# Autodesk Inventor assembly: HorizontalBit
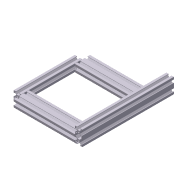
[picture p0: Inventor's stored thumbnail of the model, 180x180]
Saved by Autodesk Inventor 2014 (Build 180170000, 170)
## iProperties
Created: 2014-08-09
Part Number: HorizontalBit
Document SubType Name: Assembly
Designer: Peele
Author: Peele
## Documents named in this file (6)
- E:\Copy\DLP\Concept\SubAssem\HorizontalBit.iam
- E:\Copy\DLP\Concept\StockParts\8020-25.ipt
- E:\Copy\DLP\Concept\StockParts\8020-25-Double\8020-2505.ipt
- E:\Copy\DLP\Concept\StockParts\8020-25-Double.ipt
- E:\Copy\DLP\Concept\StockParts\8020-25\8020-2508.ipt
- E:\Copy\DLP\Concept\StockParts\8020-25-Double\8020-2507.ipt
## Components (4 placed, 3 different names)
1. 8020-2505:1 — Flush:4, Mate:4, Flush:10, Mate:5, Flush:12, Flush:13, Flush:16
2. 8020-2505:2 — Flush:4, Flush:14, Flush:17
3. 8020-2508:3 — Mate:4, Flush:10, Flush:14, Flush:16, Flush:17
4. 8020-2507:3 — Mate:5, Flush:12, Flush:13
## Relationships (9: Flush 7, Mate 2)
- Flush:4: 8020-2505:1 ↔ 8020-2505:2
- Mate:4: 8020-2505:1 ↔ 8020-2508:3
- Flush:10: 8020-2505:1 ↔ 8020-2508:3
- Mate:5: 8020-2505:1 ↔ 8020-2507:3
- Flush:12: 8020-2505:1 ↔ 8020-2507:3
- Flush:13: 8020-2505:1 ↔ 8020-2507:3
- Flush:14: 8020-2505:2 ↔ 8020-2508:3
- Flush:16 (25 mm): 8020-2505:1 ↔ 8020-2508:3
- Flush:17 (25 mm): 8020-2505:2 ↔ 8020-2508:3
